# Autodesk Inventor assembly: Time_Space_Assembled
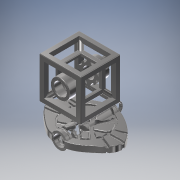
[picture p0: Inventor's stored thumbnail of the model, 180x180]
Saved by Autodesk Inventor 2019 (Build 230136000, 136)
## iProperties
Created: 2019-06-12
Part Number: Time_Space_Assembled
Document SubType Name: Assembly
Designer: Jorian Bruslind
Author: Jorian Bruslind
## Documents named in this file (3)
- C:\Users\Jorian Bruslind\Documents\GitHub\PersonalProjects\Inventor Projects\Infinity\Time_Space_Assembled.iam
- C:\Users\Jorian Bruslind\Documents\GitHub\PersonalProjects\Inventor Projects\Infinity\Agamoto.ipt
- C:\Users\Jorian Bruslind\Documents\GitHub\PersonalProjects\Inventor Projects\Infinity\Inner.ipt
## Components (2 placed, 2 different names)
1. Agamoto:1 — Flush:1, Mate:1
2. Inner:1 — Flush:1, Mate:1
## Relationships (2: Flush 1, Mate 1)
- Flush:1: Agamoto:1 ↔ Inner:1
- Mate:1 (10 mm): Agamoto:1 ↔ Inner:1
